# Autodesk Inventor assembly: EnsambleAislante
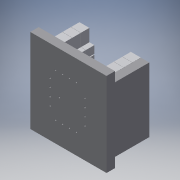
[picture p0: Inventor's stored thumbnail of the model, 180x180]
Saved by Autodesk Inventor 2017 (Build 210142000, 142)
## iProperties
Created: 2021-02-12
Part Number: EnsambleAislante
Document SubType Name: Assembly
Designer: USUARIO
Author: USUARIO
## Documents named in this file (7)
- D:\Laboratorio\Mufla\2021\Mufla 9L Psoc Artilab #0045884XX OP202139\Modelo\EnsambleAislante.iam
- D:\Laboratorio\Mufla\2021\Mufla 9L Psoc Artilab #0045884XX OP202139\Modelo\TapaFrontal.ipt
- D:\Laboratorio\Mufla\2021\Mufla 9L Psoc Artilab #0045884XX OP202139\Modelo\PiezaInferior.ipt
- D:\Laboratorio\Mufla\2021\Mufla 9L Psoc Artilab #0045884XX OP202139\Modelo\Piso.ipt
- D:\Laboratorio\Mufla\2021\Mufla 9L Psoc Artilab #0045884XX OP202139\Modelo\Lateral.ipt
- D:\Laboratorio\Mufla\2021\Mufla 9L Psoc Artilab #0045884XX OP202139\Modelo\Trasera.ipt
- D:\Laboratorio\Mufla\2021\Mufla 9L Psoc Artilab #0045884XX OP202139\Modelo\EnsambleResistencia.iam
## Components (21 placed, 6 different names)
1. TapaFrontal:1 — Mate:1, Mate:9, Mate:12, Mate:19, Flush:30, Flush:32, Flush:35, Flush:36, Flush:37
2. PiezaInferior:1 — Mate:1, Mate:2, Flush:3, Flush:29, Flush:33, Mate:31
3. Piso:1 — Flush:29, Flush:34, Flush:35
4. PiezaInferior:2 — Mate:2, Flush:3, Mate:3, Flush:5, Flush:34, Mate:30, Mate:33
5. PiezaInferior:3 — Mate:4, Flush:7, Mate:11, Mate:28
6. PiezaInferior:4 — Mate:3, Flush:5, Mate:4, Flush:7, Mate:29
7. PiezaInferior:5 — Mate:9, Mate:20, Flush:38
8. PiezaInferior:6 — Mate:14, Flush:39
9. PiezaInferior:7 — Mate:17, Mate:26, Mate:27, Flush:41
10. PiezaInferior:8 — Mate:16, Flush:40, Mate:35
11. Lateral:1 — Mate:11, Mate:12, Mate:13, Flush:19, Flush:30, Mate:31, Flush:38
12. Lateral:2 — Mate:13, Mate:14, Flush:19, Mate:15, Flush:20, Mate:30, Flush:39
13. Lateral:3 — Mate:15, Flush:20, Mate:16, Flush:21, Mate:18, Mate:29, Flush:40
14. Lateral:4 — Flush:21, Mate:17, Mate:18, Mate:28, Flush:41
15. Lateral:5 — Mate:19, Mate:20, Flush:33, Mate:32, Flush:42, Mate:36, Mate:37
16. Lateral:8 — Mate:26, Flush:32
17. Trasera:1 — Mate:27, Flush:36, Flush:37
18. Lateral:9 — Mate:32, Flush:42, Mate:33, Mate:34, Flush:43
19. Lateral:10 — Mate:34, Flush:43, Mate:35
20. EnsambleResistencia:1 [sub-assembly] — Mate:36
21. EnsambleResistencia:2 [sub-assembly] — Mate:37
## Relationships (53: Mate 30, Flush 23)
- Mate:1 (1 mm): TapaFrontal:1 ↔ PiezaInferior:1
- Mate:2 (1 mm): PiezaInferior:1 ↔ PiezaInferior:2
- Flush:3: PiezaInferior:1 ↔ PiezaInferior:2
- Mate:3 (1 mm): PiezaInferior:2 ↔ PiezaInferior:4
- Flush:5: PiezaInferior:2 ↔ PiezaInferior:4
- Mate:4 (1 mm): PiezaInferior:3 ↔ PiezaInferior:4
- Flush:7: PiezaInferior:3 ↔ PiezaInferior:4
- [Mate] (1 mm): PiezaInferior:5 ↔ PiezaInferior:6
- [Flush]: PiezaInferior:5 ↔ PiezaInferior:6
- [Mate] (1 mm): PiezaInferior:6 ↔ PiezaInferior:8
- [Flush]: PiezaInferior:6 ↔ PiezaInferior:8
- [Mate] (1 mm): PiezaInferior:7 ↔ PiezaInferior:8
- [Flush]: PiezaInferior:7 ↔ PiezaInferior:8
- Mate:9 (1 mm): TapaFrontal:1 ↔ PiezaInferior:5
- Mate:11 (1 mm): PiezaInferior:3 ↔ Lateral:1
- Mate:12 (1 mm): TapaFrontal:1 ↔ Lateral:1
- Mate:13 (1 mm): Lateral:1 ↔ Lateral:2
- Mate:14 (1 mm): PiezaInferior:6 ↔ Lateral:2
- Flush:19: Lateral:1 ↔ Lateral:2
- Mate:15 (1 mm): Lateral:2 ↔ Lateral:3
- Flush:20: Lateral:2 ↔ Lateral:3
- Mate:16 (1 mm): PiezaInferior:8 ↔ Lateral:3
- Flush:21: Lateral:3 ↔ Lateral:4
- Mate:17 (1 mm): PiezaInferior:7 ↔ Lateral:4
- Mate:18 (1 mm): Lateral:3 ↔ Lateral:4
- Mate:19 (1 mm): TapaFrontal:1 ↔ Lateral:5
- Mate:20 (1 mm): PiezaInferior:5 ↔ Lateral:5
- Mate:26 (1 mm): PiezaInferior:7 ↔ Lateral:8
- Mate:27 (1 mm): PiezaInferior:7 ↔ Trasera:1
- Flush:29: PiezaInferior:1 ↔ Piso:1
- Flush:30: TapaFrontal:1 ↔ Lateral:1
- Flush:32: TapaFrontal:1 ↔ Lateral:8
- Flush:33: PiezaInferior:1 ↔ Lateral:5
- Flush:34: Piso:1 ↔ PiezaInferior:2
- Flush:35: TapaFrontal:1 ↔ Piso:1
- Mate:28 (1 mm): PiezaInferior:3 ↔ Lateral:4
- Mate:29 (1 mm): PiezaInferior:4 ↔ Lateral:3
- Mate:30 (1 mm): PiezaInferior:2 ↔ Lateral:2
- Mate:31 (1 mm): PiezaInferior:1 ↔ Lateral:1
- Flush:36: TapaFrontal:1 ↔ Trasera:1
- Flush:37: TapaFrontal:1 ↔ Trasera:1
- Flush:38: PiezaInferior:5 ↔ Lateral:1
- Flush:39: PiezaInferior:6 ↔ Lateral:2
- Flush:40: PiezaInferior:8 ↔ Lateral:3
- Flush:41: PiezaInferior:7 ↔ Lateral:4
- Mate:32 (1 mm): Lateral:5 ↔ Lateral:9
- Flush:42: Lateral:5 ↔ Lateral:9
- Mate:33 (1 mm): PiezaInferior:2 ↔ Lateral:9
- Mate:34 (1 mm): Lateral:9 ↔ Lateral:10
- Flush:43: Lateral:9 ↔ Lateral:10
- Mate:35 (1 mm): PiezaInferior:8 ↔ Lateral:10
- Mate:36 (2 mm): Lateral:5 ↔ EnsambleResistencia:1
- Mate:37 (2 mm): Lateral:5 ↔ EnsambleResistencia:2
## Named parameters: d30_d24 = 1 mm, d32_d26 = 0 mm, d33_d18 = 1 mm, d35_d20 = 0 mm, d36_d21 = 1 mm, d38_d23 = 0 mm
